# Autodesk Inventor assembly: Gameboy NG- slim
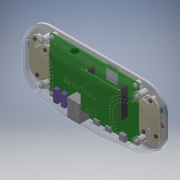
[picture p0: Inventor's stored thumbnail of the model, 180x180]
Saved by Autodesk Inventor 2019 (Build 230136000, 136)
## iProperties
Created: 2018-06-05
Part Number: Gameboy NG- slim
Material: Générique
Document SubType Name: Assembly
Designer: dimercur
Author: dimercur
## Documents named in this file (14)
- D:\Users\dimercur\Documents locaux\Travail\git\arm-ada-ng\hardware\Box\Gameboy NG- slim.iam
- D:\Users\dimercur\Documents locaux\Travail\git\arm-ada-ng\hardware\Box\STM32F746G-Disco.ipt
- D:\Users\dimercur\Documents locaux\Travail\git\arm-ada-ng\hardware\Box\Partie Haute.ipt
- D:\Users\dimercur\Documents locaux\Travail\git\arm-ada-ng\hardware\Box\Satellite Gauche.iam
- D:\Users\dimercur\Documents locaux\Travail\git\arm-ada-ng\hardware\Box\Satellite Droit.iam
- D:\Users\dimercur\Documents locaux\Travail\git\arm-ada-ng\hardware\Box\PCB Wifi.ipt
- U:\Inventor\Content Center Files\R2019\fr-FR\ISO 7045  H\ISO 7045 - M3 x 8 - 4.8 - H - ISO.ipt
- U:\Inventor\Content Center Files\R2019\fr-FR\ISO 7045  Z\ISO 7045 - M3 x 4 - 4.8 - Z - ISO.ipt
- D:\Users\dimercur\Documents locaux\Travail\git\arm-ada-ng\hardware\Box\Button-SNES.ipt
- D:\Users\dimercur\Documents locaux\Travail\git\arm-ada-ng\hardware\Box\DPAD-Gameboy.ipt
- D:\Users\dimercur\Documents locaux\Travail\git\arm-ada-ng\hardware\Box\Membrane-DPAD.ipt
- D:\Users\dimercur\Documents locaux\Travail\git\arm-ada-ng\hardware\Box\Membrane - Boutons.ipt
- D:\Users\dimercur\Documents locaux\Travail\git\arm-ada-ng\hardware\Box\Partie basse-slim.ipt
- U:\Inventor\Content Center Files\R2019\fr-FR\ISO 7045  Z\ISO 7045 - M2,5 x 5 - 4.8 - Z - ISO.ipt
## Components (27 placed, 13 different names)
1. STM32F746G-Disco:1 — Placage:1, Placage:2, Placage:3, Placage:27, Placage:28, Placage:29, Logement:11, Logement:12, Logement:13, Logement:14
2. Partie Haute:1 — Placage:1, Placage:2, Placage:3, Affleurement:1, Placage:4, Placage:31, Placage:33, Placage:39, Placage:40, Placage:43, Placage:44, Placage:45, Placage:46, Placage:47, Placage:48, Placage:49, Placage:50, Placage:52, Angle:1, Placage:55, Placage:58, Placage:59, Placage:60, Placage:61, Placage:62, Placage:63, Placage:64
3. Satellite Gauche:1 [sub-assembly] — Placage:55, Placage:63, Placage:64, Logement:15, Logement:16, Logement:17
4. Satellite Droit:1 [sub-assembly] — Placage:53, Placage:58, Placage:59, Logement:18, Logement:19, Logement:20
5. PCB Wifi:1 — Placage:27, Placage:28, Placage:29
6. ISO 7045 H M3 x 8 - 4.8 - H:1
7. ISO 7045 H M3 x 8 - 4.8 - H:2
8. ISO 7045 H M3 x 8 - 4.8 - H:3
9. ISO 7045 H M3 x 8 - 4.8 - H:4
10. ISO 7045 Z M3 x 4 - 4.8 - Z:1 — Logement:11
11. ISO 7045 Z M3 x 4 - 4.8 - Z:2 — Logement:12
12. ISO 7045 Z M3 x 4 - 4.8 - Z:3 — Logement:13
13. ISO 7045 Z M3 x 4 - 4.8 - Z:4 — Logement:14
14. Button-SNES:1 — Placage:33, Placage:48
15. Button-SNES:2 — Placage:45, Placage:49
16. Button-SNES:3 — Placage:47, Placage:50
17. Button-SNES:4 — Placage:31, Placage:46, Placage:51
18. DPAD-Gameboy:1 — Placage:39, Placage:40, Placage:41, Placage:42, Placage:43
19. Membrane-DPAD:1 — Placage:41, Placage:42, Placage:44
20. Membrane - Boutons:1 — Placage:51, Placage:52, Angle:1, Placage:53
21. Dessous - Slim:1 — Placage:60, Placage:61, Placage:62
22. ISO 7045 Z M2,5 x 5 - 4.8 - Z:1 — Logement:15
23. ISO 7045 Z M2,5 x 5 - 4.8 - Z:2 — Logement:16
24. ISO 7045 Z M2,5 x 5 - 4.8 - Z:3 — Logement:17
25. ISO 7045 Z M2,5 x 5 - 4.8 - Z:4 — Logement:18
26. ISO 7045 Z M2,5 x 5 - 4.8 - Z:5 — Logement:19
27. ISO 7045 Z M2,5 x 5 - 4.8 - Z:6 — Logement:20
## Relationships (44: Mate 32, Insert 10, Flush 1, Angle 1)
- Placage:1 [Mate]: STM32F746G-Disco:1 ↔ Partie Haute:1
- Placage:2 [Mate]: STM32F746G-Disco:1 ↔ Partie Haute:1
- Placage:3 [Mate]: STM32F746G-Disco:1 ↔ Partie Haute:1
- Affleurement:1 [Flush]: Partie Haute:1
- Placage:4 [Mate]: Partie Haute:1
- Placage:27 [Mate]: STM32F746G-Disco:1 ↔ PCB Wifi:1
- Placage:28 [Mate]: STM32F746G-Disco:1 ↔ PCB Wifi:1
- Placage:29 [Mate]: STM32F746G-Disco:1 ↔ PCB Wifi:1
- Logement:11 [Insert]: STM32F746G-Disco:1 ↔ ISO 7045 Z M3 x 4 - 4.8 - Z:1
- Logement:12 [Insert]: STM32F746G-Disco:1 ↔ ISO 7045 Z M3 x 4 - 4.8 - Z:2
- Logement:13 [Insert]: STM32F746G-Disco:1 ↔ ISO 7045 Z M3 x 4 - 4.8 - Z:3
- Logement:14 [Insert]: STM32F746G-Disco:1 ↔ ISO 7045 Z M3 x 4 - 4.8 - Z:4
- Placage:31 [Mate]: Partie Haute:1 ↔ Button-SNES:4
- Placage:33 [Mate]: Partie Haute:1 ↔ Button-SNES:1
- Placage:39 [Mate] (0.25 mm): Partie Haute:1 ↔ DPAD-Gameboy:1
- Placage:40 [Mate] (0.25 mm): Partie Haute:1 ↔ DPAD-Gameboy:1
- Placage:41 [Mate]: DPAD-Gameboy:1 ↔ Membrane-DPAD:1
- Placage:42 [Mate]: DPAD-Gameboy:1 ↔ Membrane-DPAD:1
- Placage:43 [Mate]: Partie Haute:1 ↔ DPAD-Gameboy:1
- Placage:44 [Mate]: Partie Haute:1 ↔ Membrane-DPAD:1
- Placage:45 [Mate]: Partie Haute:1 ↔ Button-SNES:2
- Placage:46 [Mate]: Partie Haute:1 ↔ Button-SNES:4
- Placage:47 [Mate]: Partie Haute:1 ↔ Button-SNES:3
- Placage:48 [Mate]: Partie Haute:1 ↔ Button-SNES:1
- Placage:49 [Mate]: Partie Haute:1 ↔ Button-SNES:2
- Placage:50 [Mate]: Partie Haute:1 ↔ Button-SNES:3
- Placage:51 [Mate]: Button-SNES:4 ↔ Membrane - Boutons:1
- Placage:52 [Mate]: Partie Haute:1 ↔ Membrane - Boutons:1
- Angle:1 (0 deg): Partie Haute:1 ↔ Membrane - Boutons:1
- Placage:53 [Mate]: Satellite Droit:1 ↔ Membrane - Boutons:1
- Placage:55 [Mate]: Partie Haute:1 ↔ Satellite Gauche:1
- Placage:58 [Mate]: Partie Haute:1 ↔ Satellite Droit:1
- Placage:59 [Mate]: Partie Haute:1 ↔ Satellite Droit:1
- Placage:60 [Mate]: Partie Haute:1 ↔ Dessous - Slim:1
- Placage:61 [Mate]: Partie Haute:1 ↔ Dessous - Slim:1
- Placage:62 [Mate]: Partie Haute:1 ↔ Dessous - Slim:1
- Placage:63 [Mate]: Partie Haute:1 ↔ Satellite Gauche:1
- Placage:64 [Mate]: Partie Haute:1 ↔ Satellite Gauche:1
- Logement:15 [Insert]: Satellite Gauche:1 ↔ ISO 7045 Z M2,5 x 5 - 4.8 - Z:1
- Logement:16 [Insert]: Satellite Gauche:1 ↔ ISO 7045 Z M2,5 x 5 - 4.8 - Z:2
- Logement:17 [Insert]: Satellite Gauche:1 ↔ ISO 7045 Z M2,5 x 5 - 4.8 - Z:3
- Logement:18 [Insert]: Satellite Droit:1 ↔ ISO 7045 Z M2,5 x 5 - 4.8 - Z:4
- Logement:19 [Insert]: Satellite Droit:1 ↔ ISO 7045 Z M2,5 x 5 - 4.8 - Z:5
- Logement:20 [Insert]: Satellite Droit:1 ↔ ISO 7045 Z M2,5 x 5 - 4.8 - Z:6
